# Autodesk Inventor assembly: Drive Constraints
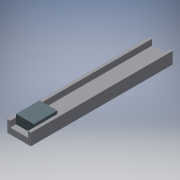
[picture p0: Inventor's stored thumbnail of the model, 180x180]
Saved by Autodesk Inventor 2019 Beta2 (Build 230110000, 110) ContinuousBuild 0
## iProperties
Created: 2014-03-12
Part Number: Drive Constraints
Document SubType Name: Assembly
Designer: John
Author: John
## Documents named in this file (3)
- C:\Users\helfenj\Desktop\Ex_Files_Autodesk_Inventor_2019_EssT\Exercise Files\14_Using constraints to position parts\14_04\Drive Constraints.iam
- C:\Users\helfenj\Desktop\Ex_Files_Autodesk_Inventor_2019_EssT\Exercise Files\14_Using constraints to position parts\14_04\Base.ipt
- C:\Users\helfenj\Desktop\Ex_Files_Autodesk_Inventor_2019_EssT\Exercise Files\14_Using constraints to position parts\14_04\Slide.ipt
## Components (2 placed, 2 different names)
1. Base:1 — Mate:1, Mate:2
2. Slide:1 — Mate:1, Mate:2
## Relationships (2: Mate 2)
- Mate:1: Base:1 ↔ Slide:1
- Mate:2: Base:1 ↔ Slide:1
